# Autodesk Inventor assembly: Assem1
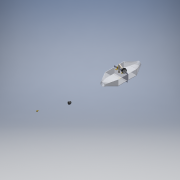
[picture p0: Inventor's stored thumbnail of the model, 180x180]
Saved by Autodesk Inventor 2017 (Build 210142000, 142)
## iProperties
Created: 2014-08-02
Part Number: Assem1
Document SubType Name: Assembly
Designer: XuZhiqing
Sending System: SolidWorks 2014
Last Author: 1
Last Saved: 2014-09-23
Author: XuZhiqing
## Documents named in this file (9)
- C:\Users\XuZhiqing\Desktop\Project01-CFD_the_sys\CAD-Whole Sys\filter and gauge\gas pressure gauge\gas pressure gauge.iam
- C:\Users\XuZhiqing\Desktop\Project01-CFD_the_sys\CAD-Whole Sys\filter and gauge\gas pressure gauge\Part8.ipt
- C:\Users\XuZhiqing\Desktop\Project01-CFD_the_sys\CAD-Whole Sys\filter and gauge\gas pressure gauge\Part10.ipt
- C:\Users\XuZhiqing\Desktop\Project01-CFD_the_sys\CAD-Whole Sys\filter and gauge\gas pressure gauge\Part19.ipt
- C:\Users\XuZhiqing\Desktop\Project01-CFD_the_sys\CAD-Whole Sys\filter and gauge\gas pressure gauge\Part21.ipt
- C:\Users\XuZhiqing\Desktop\Project01-CFD_the_sys\CAD-Whole Sys\filter and gauge\gas pressure gauge\Solid5.ipt
- C:\Users\XuZhiqing\Desktop\Project01-CFD_the_sys\CAD-Whole Sys\filter and gauge\gas pressure gauge\gauge3.ipt
- C:\Users\XuZhiqing\Desktop\Project01-CFD_the_sys\CAD-Whole Sys\filter and gauge\gas pressure gauge\Solid9.ipt
- C:\Users\XuZhiqing\Desktop\Project01-CFD_the_sys\CAD-Whole Sys\filter and gauge\filter\Assem1.iam
## Components (9 placed, 8 different names)
1. Part8:1
2. Part10:1 — Mate:2, Mate:3, Mate:4, Mate:5
3. Part19:1 — Mate:4, Mate:5, Mate:7, Mate:8
4. Part21:1 — Mate:1, Mate:2, Mate:3
5. Solid5:1
6. gauge3:1 — Mate:9, Mate:10
7. Solid9:1
8. Assem1:1 [sub-assembly] — Mate:1
9. Part10:2 — Mate:7, Mate:8, Mate:9, Mate:10
## Relationships (9: Mate 9)
- Mate:1: Part21:1 ↔ Assem1:1
- Mate:2: Part10:1 ↔ Part21:1
- Mate:3: Part10:1 ↔ Part21:1
- Mate:4: Part10:1 ↔ Part19:1
- Mate:5: Part10:1 ↔ Part19:1
- Mate:7: Part19:1 ↔ Part10:2
- Mate:8: Part19:1 ↔ Part10:2
- Mate:9: gauge3:1 ↔ Part10:2
- Mate:10: gauge3:1 ↔ Part10:2
